# Autodesk Inventor assembly: BallBot_macro
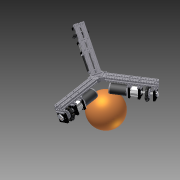
[picture p0: Inventor's stored thumbnail of the model, 180x180]
Saved by Autodesk Inventor 2012 (Build 160160000, 160)
## iProperties
Created: 2012-10-25
Part Number: BallBot_macro
Document SubType Name: Assembly
Designer: Andrew G. Meyer
Author: Andrew G. Meyer
## Documents named in this file (7)
- C:\Users\Andrew G. Meyer\Documents\Projects\BallBot\macro\CAD\BallBot_macro.iam
- C:\Users\Andrew G. Meyer\Documents\Projects\BallBot\macro\CAD\Drivetrain_Module.iam
- C:\Users\Andrew G. Meyer\Documents\Projects\BallBot\macro\CAD\drive_frame_bracket.ipt
- C:\Users\Andrew G. Meyer\Documents\Projects\BallBot\macro\CAD\drive_frame_endpiece.iam
- C:\Users\Andrew G. Meyer\Documents\Inventor\Content Center Files\R2012\en-US\ANSI B18.3(05)\ANSI B18.3 - 1_4-20 UNC - 0.5(31).ipt
- C:\Users\Andrew G. Meyer\Documents\Inventor\Content Center Files\R2012\en-US\ANSI B18.3(05)\ANSI B18.3 - 1_4-20 UNC - 1.5(31).ipt
- C:\Users\Andrew G. Meyer\Documents\Projects\BallBot\macro\CAD\BasketBall.ipt
## Components (22 placed, 6 different names)
1. Drivetrain_Module:1 [sub-assembly] — Mate:13, Mate:14, Mate:15, Mate:22
2. Drivetrain_Module:2 [sub-assembly] — Mate:19, Mate:20, Mate:21, Tangent:2
3. Drivetrain_Module:3 [sub-assembly] — Mate:16, Mate:17, Mate:18, Tangent:1
4. drive_frame_bracket:1 — Mate:4, Mate:5, Mate:10, Mate:12, Insert:5, Insert:6
5. drive_frame_bracket:2 — Mate:2, Mate:6, Mate:7, Mate:11, Insert:3, Insert:4
6. drive_frame_bracket:3 — Mate:1, Mate:3, Mate:8, Mate:9, Insert:1, Insert:2
7. drive_frame_endpiece:1 [sub-assembly] — Mate:1, Mate:2, Mate:7, Mate:8, Mate:19, Mate:20, Mate:21, Insert:7, Insert:8
8. drive_frame_endpiece:2 [sub-assembly] — Mate:3, Mate:4, Mate:9, Mate:10, Mate:16, Mate:17, Mate:18, Insert:9, Insert:10
9. drive_frame_endpiece:3 [sub-assembly] — Mate:5, Mate:6, Mate:11, Mate:12, Mate:13, Mate:14, Mate:15, Insert:11, Insert:12
10. Hexagon Socket Head Cap Screw - Inch 1/4 - 20 UNC - 1/2:1 — Insert:1
11. Hexagon Socket Head Cap Screw - Inch 1/4 - 20 UNC - 1/2:2 — Insert:2
12. Hexagon Socket Head Cap Screw - Inch 1/4 - 20 UNC - 1/2:3 — Insert:4
13. Hexagon Socket Head Cap Screw - Inch 1/4 - 20 UNC - 1/2:4 — Insert:6
14. Hexagon Socket Head Cap Screw - Inch 1/4 - 20 UNC - 1/2:5 — Insert:3
15. Hexagon Socket Head Cap Screw - Inch 1/4 - 20 UNC - 1/2:6 — Insert:5
16. Hexagon Socket Head Cap Screw - Inch 1/4 - 20 UNC - 1 1/2:1 — Insert:7
17. Hexagon Socket Head Cap Screw - Inch 1/4 - 20 UNC - 1 1/2:2 — Insert:9
18. Hexagon Socket Head Cap Screw - Inch 1/4 - 20 UNC - 1 1/2:3 — Insert:11
19. Hexagon Socket Head Cap Screw - Inch 1/4 - 20 UNC - 1 1/2:4 — Insert:8
20. Hexagon Socket Head Cap Screw - Inch 1/4 - 20 UNC - 1 1/2:5 — Insert:10
21. Hexagon Socket Head Cap Screw - Inch 1/4 - 20 UNC - 1 1/2:6 — Insert:12
22. BasketBall:1 — Mate:22, Tangent:1, Tangent:2
## Relationships (36: Mate 22, Insert 12, Tangent 2)
- Mate:1: drive_frame_bracket:3 ↔ drive_frame_endpiece:1
- Mate:2: drive_frame_bracket:2 ↔ drive_frame_endpiece:1
- Mate:3: drive_frame_bracket:3 ↔ drive_frame_endpiece:2
- Mate:4: drive_frame_bracket:1 ↔ drive_frame_endpiece:2
- Mate:5: drive_frame_bracket:1 ↔ drive_frame_endpiece:3
- Mate:6: drive_frame_bracket:2 ↔ drive_frame_endpiece:3
- Mate:7: drive_frame_bracket:2 ↔ drive_frame_endpiece:1
- Mate:8: drive_frame_bracket:3 ↔ drive_frame_endpiece:1
- Mate:9: drive_frame_bracket:3 ↔ drive_frame_endpiece:2
- Mate:10: drive_frame_bracket:1 ↔ drive_frame_endpiece:2
- Mate:11: drive_frame_bracket:2 ↔ drive_frame_endpiece:3
- Mate:12: drive_frame_bracket:1 ↔ drive_frame_endpiece:3
- Insert:1: drive_frame_bracket:3 ↔ Hexagon Socket Head Cap Screw - Inch 1/4 - 20 UNC - 1/2:1
- Insert:2: drive_frame_bracket:3 ↔ Hexagon Socket Head Cap Screw - Inch 1/4 - 20 UNC - 1/2:2
- Insert:3: drive_frame_bracket:2 ↔ Hexagon Socket Head Cap Screw - Inch 1/4 - 20 UNC - 1/2:5
- Insert:4: drive_frame_bracket:2 ↔ Hexagon Socket Head Cap Screw - Inch 1/4 - 20 UNC - 1/2:3
- Insert:5: drive_frame_bracket:1 ↔ Hexagon Socket Head Cap Screw - Inch 1/4 - 20 UNC - 1/2:6
- Insert:6: drive_frame_bracket:1 ↔ Hexagon Socket Head Cap Screw - Inch 1/4 - 20 UNC - 1/2:4
- Mate:13: Drivetrain_Module:1 ↔ drive_frame_endpiece:3
- Mate:14: Drivetrain_Module:1 ↔ drive_frame_endpiece:3
- Mate:15: Drivetrain_Module:1 ↔ drive_frame_endpiece:3
- Mate:16: Drivetrain_Module:3 ↔ drive_frame_endpiece:2
- Mate:17: Drivetrain_Module:3 ↔ drive_frame_endpiece:2
- Mate:18: Drivetrain_Module:3 ↔ drive_frame_endpiece:2
- Mate:19: Drivetrain_Module:2 ↔ drive_frame_endpiece:1
- Mate:20: Drivetrain_Module:2 ↔ drive_frame_endpiece:1
- Mate:21: Drivetrain_Module:2 ↔ drive_frame_endpiece:1
- Insert:7: drive_frame_endpiece:1 ↔ Hexagon Socket Head Cap Screw - Inch 1/4 - 20 UNC - 1 1/2:1
- Insert:8: drive_frame_endpiece:1 ↔ Hexagon Socket Head Cap Screw - Inch 1/4 - 20 UNC - 1 1/2:4
- Insert:9: drive_frame_endpiece:2 ↔ Hexagon Socket Head Cap Screw - Inch 1/4 - 20 UNC - 1 1/2:2
- Insert:10: drive_frame_endpiece:2 ↔ Hexagon Socket Head Cap Screw - Inch 1/4 - 20 UNC - 1 1/2:5
- Insert:11: drive_frame_endpiece:3 ↔ Hexagon Socket Head Cap Screw - Inch 1/4 - 20 UNC - 1 1/2:3
- Insert:12: drive_frame_endpiece:3 ↔ Hexagon Socket Head Cap Screw - Inch 1/4 - 20 UNC - 1 1/2:6
- Mate:22: Drivetrain_Module:1 ↔ BasketBall:1
- Tangent:1: Drivetrain_Module:3 ↔ BasketBall:1
- Tangent:2: Drivetrain_Module:2 ↔ BasketBall:1
